# Autodesk Inventor assembly: dtmotorgearsdeadaxle
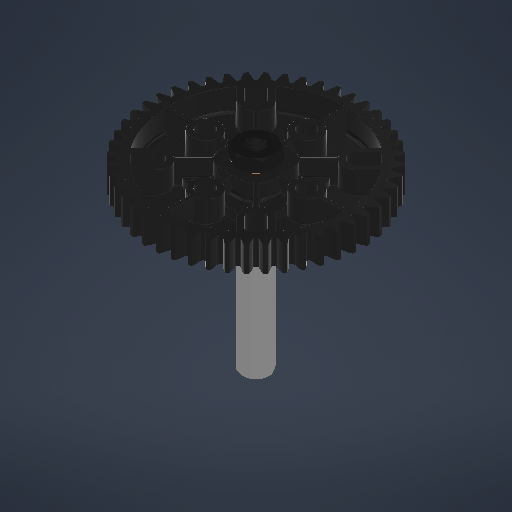
[picture p0: Inventor's stored thumbnail of the model, 512x512]
Saved by Autodesk Inventor 2026.1 (Build 301233000, 233)
## iProperties
Created: 2025-08-03
Part Number: dtmotorgearsdeadaxle
Document SubType Name: Assembly
Designer: roejo
Author: roejo
## Documents named in this file (10)
- C:\Users\roejo\OneDrive\Documents\2026WorldChampionRobot\Robots\Worlds\Subassemblies\dtmotorgearsdeadaxle -48t.iam
- C:\Users\roejo\OneDrive\Documents\2026WorldChampionRobot\Library\VEX-CAD-Inventor-1.4.2\Motion\Spacers\Washer Teflon\TWasher .375 OD x .06250.ipt
- C:\Users\roejo\OneDrive\Documents\2026WorldChampionRobot\Library\VEX-CAD-Inventor-1.4.2\Motion\Spacers\Washer Teflon.ipt
- C:\Users\roejo\OneDrive\Documents\2026WorldChampionRobot\Library\VEX-CAD-Inventor-1.4.2\Structure\Hardware\alu_nylock.ipt
- C:\Users\roejo\OneDrive\Documents\2026WorldChampionRobot\Library\VEX-CAD-Inventor-1.4.2\Structure\Standoff\Standoff 1.00.ipt
- C:\Users\roejo\OneDrive\Documents\2026WorldChampionRobot\Library\VEX-CAD-Inventor-1.4.2\Structure\Standoff.ipt
- C:\Users\roejo\OneDrive\Documents\2026WorldChampionRobot\Library\VEX-CAD-Inventor-1.4.2\Motion\Spacers\thinspacer0.25.ipt
- C:\Users\roejo\OneDrive\Documents\2026WorldChampionRobot\Library\VEX-CAD-Inventor-1.4.2\Motion\Gears\HS Gear\halfcut-48t-gear.iam
- C:\Users\roejo\OneDrive\Documents\2026WorldChampionRobot\Library\VEX-CAD-Inventor-1.4.2\Structure\Hardware\Nut Nylon\Nut Nylon - Black.ipt
- C:\Users\roejo\OneDrive\Documents\2026WorldChampionRobot\Library\VEX-CAD-Inventor-1.4.2\Structure\Hardware\Nut Nylon.ipt
## Components (6 placed, 6 different names)
1. halfcut-48t-gear:1 [sub-assembly] — Insert:5, Insert:7
2. Nut Nylon - Black:1 — Insert:5
3. Standoff 1.00:2 — Insert:6
4. alu_nylock:2 — Insert:6, Insert:9
5. TWasher .375 OD x .06250:2 — Insert:7, Insert:8
6. thinspacer0.25:2 — Insert:8, Insert:9
## Relationships (5: Insert 5)
- Insert:5: halfcut-48t-gear:1 ↔ Nut Nylon - Black:1
- Insert:6: Standoff 1.00:2 ↔ alu_nylock:2
- Insert:7 (-6.35 mm): halfcut-48t-gear:1 ↔ TWasher .375 OD x .06250:2
- Insert:8: TWasher .375 OD x .06250:2 ↔ thinspacer0.25:2
- Insert:9: alu_nylock:2 ↔ thinspacer0.25:2
